# Autodesk Inventor assembly: Block CAM Assembly
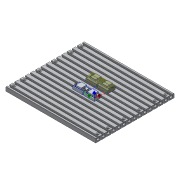
[picture p0: Inventor's stored thumbnail of the model, 180x180]
Saved by Autodesk Inventor 2016 (Build 200138000, 138)
## iProperties
Created: 2015-08-21
Part Number: Block CAM Assembly
Document SubType Name: Assembly
## Documents named in this file (7)
- E:\GitHub\CNC-Router_Accessories\Block CAM Assembly.iam
- E:\GitHub\CNC-Router_Accessories\Clamping Block.ipt
- E:\GitHub\CNC-Router_Accessories\Holding Block.ipt
- E:\GitHub\CNC-Router\T-Nutenplatte.ipt
- E:\GitHub\Standard-Parts\Zyl-Schr_ISO 4762 - M6 x 20_St-Vzkt.ipt
- E:\GitHub\Standard-Parts\U-Scheibe_ISO 7089 - 6 - 140 HV_St-Vzkt.ipt
- E:\GitHub\CNC-Router_Accessories\Jaw.ipt
## Components (23 placed, 6 different names)
1. Clamping Block:1 — Mate:1, Mate:2, Flush:1, Mate:7, Mate:8, Mate:23, Mate:24, Mate:26, Mate:27, Mate:33, Flush:5, Flush:8, Mate:34
2. Holding Block:1 — Mate:5, Mate:6, Mate:13, Mate:14, Mate:17, Mate:18, Flush:3, Flush:4, Mate:25, Flush:7
3. Clamping Block:2 — Mate:3, Mate:4, Flush:2, Mate:9, Mate:10, Mate:21, Mate:22, Mate:28, Mate:29, Mate:32, Flush:5, Flush:7
4. Holding Block:2 — Mate:11, Mate:12, Mate:15, Mate:16, Mate:19, Mate:20, Flush:3, Flush:4, Mate:25, Mate:30, Mate:31, Flush:8, Mate:34
5. T-Nutenplatte:1 — Mate:30, Mate:31, Mate:32, Mate:33
6. Zyl-Schr_ISO 4762 - M6 x 20_St-Vzkt:1 — Mate:21, Mate:29
7. U-Scheibe_ISO 7089 - 6 - 140 HV_St-Vzkt:1 — Mate:9
8. Zyl-Schr_ISO 4762 - M6 x 20_St-Vzkt:2 — Mate:14, Mate:18
9. U-Scheibe_ISO 7089 - 6 - 140 HV_St-Vzkt:2 — Mate:6
10. Zyl-Schr_ISO 4762 - M6 x 20_St-Vzkt:3 — Mate:22, Mate:28
11. U-Scheibe_ISO 7089 - 6 - 140 HV_St-Vzkt:3 — Mate:10
12. Zyl-Schr_ISO 4762 - M6 x 20_St-Vzkt:4 — Mate:13, Mate:17
13. U-Scheibe_ISO 7089 - 6 - 140 HV_St-Vzkt:4 — Mate:5
14. Zyl-Schr_ISO 4762 - M6 x 20_St-Vzkt:5 — Mate:24, Mate:26
15. U-Scheibe_ISO 7089 - 6 - 140 HV_St-Vzkt:5 — Mate:7
16. Zyl-Schr_ISO 4762 - M6 x 20_St-Vzkt:6 — Mate:23, Mate:27
17. U-Scheibe_ISO 7089 - 6 - 140 HV_St-Vzkt:6 — Mate:8
18. Zyl-Schr_ISO 4762 - M6 x 20_St-Vzkt:7 — Mate:16, Mate:19
19. U-Scheibe_ISO 7089 - 6 - 140 HV_St-Vzkt:7 — Mate:12
20. Zyl-Schr_ISO 4762 - M6 x 20_St-Vzkt:8 — Mate:15, Mate:20
21. U-Scheibe_ISO 7089 - 6 - 140 HV_St-Vzkt:8 — Mate:11
22. Jaw:1 — Mate:3, Mate:4, Flush:2
23. Jaw:2 — Mate:1, Mate:2, Flush:1
## Relationships (49: Mate 34, Insert 8, Flush 7)
- [Insert]: Zyl-Schr_ISO 4762 - M6 x 20_St-Vzkt:1 ↔ U-Scheibe_ISO 7089 - 6 - 140 HV_St-Vzkt:1
- [Insert]: Zyl-Schr_ISO 4762 - M6 x 20_St-Vzkt:2 ↔ U-Scheibe_ISO 7089 - 6 - 140 HV_St-Vzkt:2
- [Insert]: Zyl-Schr_ISO 4762 - M6 x 20_St-Vzkt:3 ↔ U-Scheibe_ISO 7089 - 6 - 140 HV_St-Vzkt:3
- [Insert]: Zyl-Schr_ISO 4762 - M6 x 20_St-Vzkt:4 ↔ U-Scheibe_ISO 7089 - 6 - 140 HV_St-Vzkt:4
- [Insert]: Zyl-Schr_ISO 4762 - M6 x 20_St-Vzkt:5 ↔ U-Scheibe_ISO 7089 - 6 - 140 HV_St-Vzkt:5
- [Insert]: Zyl-Schr_ISO 4762 - M6 x 20_St-Vzkt:6 ↔ U-Scheibe_ISO 7089 - 6 - 140 HV_St-Vzkt:6
- [Insert]: Zyl-Schr_ISO 4762 - M6 x 20_St-Vzkt:7 ↔ U-Scheibe_ISO 7089 - 6 - 140 HV_St-Vzkt:7
- [Insert]: Zyl-Schr_ISO 4762 - M6 x 20_St-Vzkt:8 ↔ U-Scheibe_ISO 7089 - 6 - 140 HV_St-Vzkt:8
- Mate:1: Clamping Block:1 ↔ Jaw:2
- Mate:2: Clamping Block:1 ↔ Jaw:2
- Flush:1: Clamping Block:1 ↔ Jaw:2
- Mate:3: Clamping Block:2 ↔ Jaw:1
- Mate:4: Clamping Block:2 ↔ Jaw:1
- Flush:2: Clamping Block:2 ↔ Jaw:1
- Mate:5: Holding Block:1 ↔ U-Scheibe_ISO 7089 - 6 - 140 HV_St-Vzkt:4
- Mate:6: Holding Block:1 ↔ U-Scheibe_ISO 7089 - 6 - 140 HV_St-Vzkt:2
- Mate:7: Clamping Block:1 ↔ U-Scheibe_ISO 7089 - 6 - 140 HV_St-Vzkt:5
- Mate:8: Clamping Block:1 ↔ U-Scheibe_ISO 7089 - 6 - 140 HV_St-Vzkt:6
- Mate:9: Clamping Block:2 ↔ U-Scheibe_ISO 7089 - 6 - 140 HV_St-Vzkt:1
- Mate:10: Clamping Block:2 ↔ U-Scheibe_ISO 7089 - 6 - 140 HV_St-Vzkt:3
- Mate:11: Holding Block:2 ↔ U-Scheibe_ISO 7089 - 6 - 140 HV_St-Vzkt:8
- Mate:12: Holding Block:2 ↔ U-Scheibe_ISO 7089 - 6 - 140 HV_St-Vzkt:7
- Mate:13 (-6 mm): Holding Block:1 ↔ Zyl-Schr_ISO 4762 - M6 x 20_St-Vzkt:4
- Mate:14 (-6 mm): Holding Block:1 ↔ Zyl-Schr_ISO 4762 - M6 x 20_St-Vzkt:2
- Mate:15 (-6 mm): Holding Block:2 ↔ Zyl-Schr_ISO 4762 - M6 x 20_St-Vzkt:8
- Mate:16 (-6 mm): Holding Block:2 ↔ Zyl-Schr_ISO 4762 - M6 x 20_St-Vzkt:7
- Mate:17 (-3.75 mm): Holding Block:1 ↔ Zyl-Schr_ISO 4762 - M6 x 20_St-Vzkt:4
- Mate:18 (-3.75 mm): Holding Block:1 ↔ Zyl-Schr_ISO 4762 - M6 x 20_St-Vzkt:2
- Mate:19 (-3.75 mm): Holding Block:2 ↔ Zyl-Schr_ISO 4762 - M6 x 20_St-Vzkt:7
- Mate:20 (-3.75 mm): Holding Block:2 ↔ Zyl-Schr_ISO 4762 - M6 x 20_St-Vzkt:8
- Mate:21 (-6 mm): Clamping Block:2 ↔ Zyl-Schr_ISO 4762 - M6 x 20_St-Vzkt:1
- Mate:22 (-6 mm): Clamping Block:2 ↔ Zyl-Schr_ISO 4762 - M6 x 20_St-Vzkt:3
- Mate:23 (-6 mm): Clamping Block:1 ↔ Zyl-Schr_ISO 4762 - M6 x 20_St-Vzkt:6
- Mate:24 (-6 mm): Clamping Block:1 ↔ Zyl-Schr_ISO 4762 - M6 x 20_St-Vzkt:5
- Flush:3: Holding Block:1 ↔ Holding Block:2
- Flush:4: Holding Block:1 ↔ Holding Block:2
- Mate:25 (5 mm): Holding Block:1 ↔ Holding Block:2
- Mate:26 (-8 mm): Clamping Block:1 ↔ Zyl-Schr_ISO 4762 - M6 x 20_St-Vzkt:5
- Mate:27 (-8 mm): Clamping Block:1 ↔ Zyl-Schr_ISO 4762 - M6 x 20_St-Vzkt:6
- Mate:28 (-8 mm): Clamping Block:2 ↔ Zyl-Schr_ISO 4762 - M6 x 20_St-Vzkt:3
- Mate:29 (-8 mm): Clamping Block:2 ↔ Zyl-Schr_ISO 4762 - M6 x 20_St-Vzkt:1
- Mate:30: Holding Block:2 ↔ T-Nutenplatte:1
- Mate:31: Holding Block:2 ↔ T-Nutenplatte:1
- Mate:32: Clamping Block:2 ↔ T-Nutenplatte:1
- Mate:33: Clamping Block:1 ↔ T-Nutenplatte:1
- Flush:5: Clamping Block:1 ↔ Clamping Block:2
- Flush:7: Holding Block:1 ↔ Clamping Block:2
- Flush:8: Clamping Block:1 ↔ Holding Block:2
- Mate:34 (30 mm): Clamping Block:1 ↔ Holding Block:2
## Named parameters: d13_d12 = 0 mm, d13_d13_d12 = 0 mm, d14_d13_d12 = 0 mm, d15_d13_d12 = 0 mm, d16_d13_d12 = 0 mm, d17_d13_d12 = 0 mm, d18_d13_d12 = 0 mm, d19_d13_d12 = 0 mm
